# Autodesk Inventor assembly: お盆完成予定1
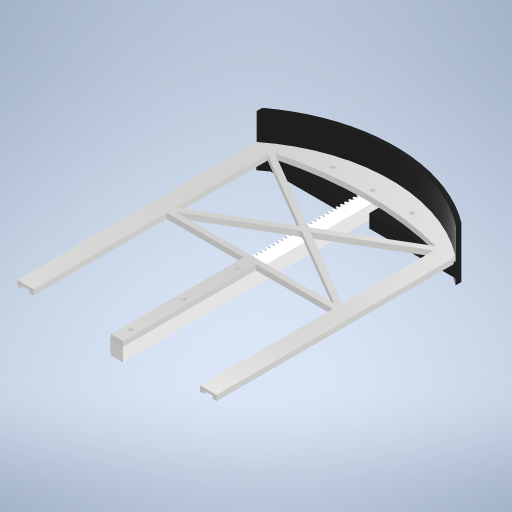
[picture p0: Inventor's stored thumbnail of the model, 512x512]
Saved by Autodesk Inventor 2023 (Build 270158000, 158)
## iProperties
Created: 2022-12-04
Part Number: お盆完成予定1
Document SubType Name: Assembly
Designer: RiSA
Author: RiSA
## Documents named in this file (4)
- E:\ロボ創\お盆試作2\お盆完成予定1.iam
- E:\ロボ創\お盆試作2\中間台2.ipt
- E:\ロボ創\お盆試作2\お盆4.ipt
- E:\ロボ創\お盆試作2\ラックM1‗8.ipt
## Components (3 placed, 3 different names)
1. 中間台2:1 — メイト:1, メイト:2, メイト:3
2. お盆4:1 — メイト:1, メイト:2, メイト:3, メイト:4, メイト:5, メイト:6
3. ラックM1‗8:1 — メイト:4, メイト:5, メイト:6
## Relationships (6: Mate 6)
- メイト:1 [Mate]: 中間台2:1 ↔ お盆4:1
- メイト:2 [Mate]: 中間台2:1 ↔ お盆4:1
- メイト:3 [Mate]: 中間台2:1 ↔ お盆4:1
- メイト:4 [Mate]: お盆4:1 ↔ ラックM1‗8:1
- メイト:5 [Mate]: お盆4:1 ↔ ラックM1‗8:1
- メイト:6 [Mate]: お盆4:1 ↔ ラックM1‗8:1
